# Autodesk Inventor assembly: np32hs
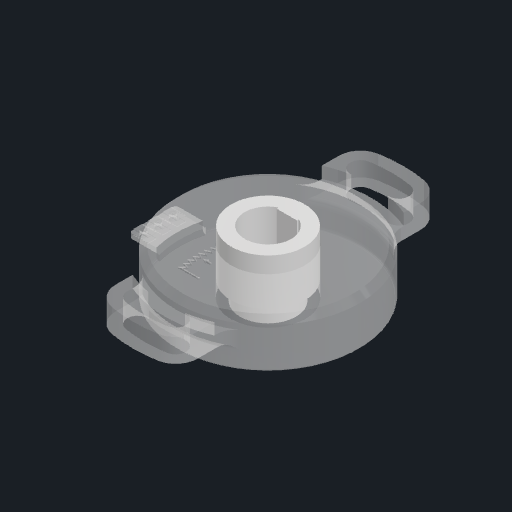
[picture p0: Inventor's stored thumbnail of the model, 512x512]
Saved by Autodesk Inventor 2025.2 (Build 292293000, 293)
## iProperties
Created: 2019-08-13
Part Number: np32hs
Document SubType Name: Assembly
Designer: valer
Preprocessor: ST-DEVELOPER v15
Title: np32hs
Revision Number: AFirst version
## Documents named in this file (3)
- C:\Users\valer\Desktop\str1ker\cad\external\np32hs.iam
- C:\Users\valer\Desktop\str1ker\cad\external\Np32HS part_Standard1_Standard.ipt
- C:\Users\valer\Desktop\str1ker\cad\external\Part6.ipt
## Components (2 placed, 2 different names)
1. Np32HS part_Standard1_Standard — Mate:1, Angle:1
2. Part6 — Mate:1
## Relationships (2: Mate 1, Angle 1)
- Mate:1: Np32HS part_Standard1_Standard ↔ Part6
- Angle:1 (0 deg): Np32HS part_Standard1_Standard
